# Autodesk Inventor assembly: robot_2016
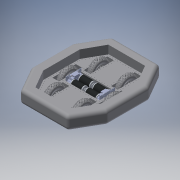
[picture p0: Inventor's stored thumbnail of the model, 180x180]
Saved by Autodesk Inventor 2016 (Build 200138000, 138)
## iProperties
Created: 2016-02-01
Part Number: robot_2016
Document SubType Name: Assembly
Designer: Mentor1102
Sending System: CREO PARAMETRIC BY PTC INC, 2014440
Preprocessor: CREO PARAMETRIC BY PTC INC, 2014440
Title: ROBOT2_ASM
Author: folkj_000
Revision Number: 24LAST_VERSION
## Documents named in this file (52)
- C:\Users\Mentor1102\Desktop\4901 CAD\RobotBase2016\robot_2016.iam
- C:\Users\Mentor1102\Desktop\4901 CAD\RobotBase2016\TOP_PLATE2_AF0.ipt
- C:\Users\Mentor1102\Desktop\4901 CAD\RobotBase2016\MOTORMOUNTBAR_AF0.ipt
- C:\Users\Mentor1102\Desktop\4901 CAD\RobotBase2016\MOTORMOUNTBAR_AF1.ipt
- C:\Users\Mentor1102\Desktop\4901 CAD\RobotBase2016\217-2642-STEP-20140807_AF0.ipt
- C:\Users\Mentor1102\Desktop\4901 CAD\RobotBase2016\217-2642-STEP-20140807_AF1.ipt
- C:\Users\Mentor1102\Desktop\4901 CAD\RobotBase2016\FR8ZZ_HEX_BEARING_1_AF0.ipt
- C:\Users\Mentor1102\Desktop\4901 CAD\RobotBase2016\FR8ZZ_HEX_BEARING_1_AF1.ipt
- C:\Users\Mentor1102\Desktop\4901 CAD\RobotBase2016\PNEUMATIC_WHEEL_AF0_ASM.iam
- C:\Users\Mentor1102\Desktop\4901 CAD\RobotBase2016\AM-1305_500_HEX_SPACER_1_AF0.ipt
- C:\Users\Mentor1102\Desktop\4901 CAD\RobotBase2016\217-2642-STEP-20140807_AF2.ipt
- C:\Users\Mentor1102\Desktop\4901 CAD\RobotBase2016\FR8ZZ_HEX_BEARING_1_AF2.ipt
- C:\Users\Mentor1102\Desktop\4901 CAD\RobotBase2016\FR8ZZ_HEX_BEARING_1_AF3.ipt
- C:\Users\Mentor1102\Desktop\4901 CAD\RobotBase2016\PNEUMATIC_WHEEL_AF1_ASM.iam
- C:\Users\Mentor1102\Desktop\4901 CAD\RobotBase2016\AM-1305_500_HEX_SPACER_1_AF1.ipt
- C:\Users\Mentor1102\Desktop\4901 CAD\RobotBase2016\217-2642-STEP-20140807_AF3.ipt
- C:\Users\Mentor1102\Desktop\4901 CAD\RobotBase2016\PNEUMATIC_WHEEL_AF2_ASM.iam
- C:\Users\Mentor1102\Desktop\4901 CAD\RobotBase2016\AM-1305_500_HEX_SPACER_1_AF2.ipt
- C:\Users\Mentor1102\Desktop\4901 CAD\RobotBase2016\217-2642-STEP-20140807_AF4.ipt
- C:\Users\Mentor1102\Desktop\4901 CAD\RobotBase2016\3X1_9_AF0.ipt
- C:\Users\Mentor1102\Desktop\4901 CAD\RobotBase2016\3X1_9_AF1.ipt
- C:\Users\Mentor1102\Desktop\4901 CAD\RobotBase2016\217-2642-STEP-20140807_AF5.ipt
- C:\Users\Mentor1102\Desktop\4901 CAD\RobotBase2016\217-2642-STEP-20140807_AF6.ipt
- C:\Users\Mentor1102\Desktop\4901 CAD\RobotBase2016\FR8ZZ_HEX_BEARING_1_AF4.ipt
- C:\Users\Mentor1102\Desktop\4901 CAD\RobotBase2016\FR8ZZ_HEX_BEARING_1_AF5.ipt
- C:\Users\Mentor1102\Desktop\4901 CAD\RobotBase2016\PNEUMATIC_WHEEL_AF3_ASM.iam
- C:\Users\Mentor1102\Desktop\4901 CAD\RobotBase2016\AM-1305_500_HEX_SPACER_1_AF3.ipt
- C:\Users\Mentor1102\Desktop\4901 CAD\RobotBase2016\217-2642-STEP-20140807_AF7.ipt
- C:\Users\Mentor1102\Desktop\4901 CAD\RobotBase2016\FR8ZZ_HEX_BEARING_1_AF6.ipt
- C:\Users\Mentor1102\Desktop\4901 CAD\RobotBase2016\FR8ZZ_HEX_BEARING_1_AF7.ipt
- C:\Users\Mentor1102\Desktop\4901 CAD\RobotBase2016\PNEUMATIC_WHEEL_AF4_ASM.iam
- C:\Users\Mentor1102\Desktop\4901 CAD\RobotBase2016\AM-1305_500_HEX_SPACER_1_AF4.ipt
- C:\Users\Mentor1102\Desktop\4901 CAD\RobotBase2016\217-2642-STEP-20140807_AF8.ipt
- C:\Users\Mentor1102\Desktop\4901 CAD\RobotBase2016\PNEUMATIC_WHEEL_AF5_ASM.iam
- C:\Users\Mentor1102\Desktop\4901 CAD\RobotBase2016\AM-1305_500_HEX_SPACER_1_AF5.ipt
- C:\Users\Mentor1102\Desktop\4901 CAD\RobotBase2016\217-2642-STEP-20140807_AF9.ipt
- C:\Users\Mentor1102\Desktop\4901 CAD\RobotBase2016\BAR2_18IN_AF0.ipt
- C:\Users\Mentor1102\Desktop\4901 CAD\RobotBase2016\BAR2_18IN_AF1.ipt
- C:\Users\Mentor1102\Desktop\4901 CAD\RobotBase2016\BAR1_AF0.ipt
- C:\Users\Mentor1102\Desktop\4901 CAD\RobotBase2016\BAR1_AF1.ipt
- C:\Users\Mentor1102\Desktop\4901 CAD\RobotBase2016\BAR6_FRONT_AF0.ipt
- C:\Users\Mentor1102\Desktop\4901 CAD\RobotBase2016\BAR1_AF2.ipt
- C:\Users\Mentor1102\Desktop\4901 CAD\RobotBase2016\BAR1_AF3.ipt
- C:\Users\Mentor1102\Desktop\4901 CAD\RobotBase2016\BAR6_FRONT_AF1.ipt
- C:\Users\Mentor1102\Desktop\4901 CAD\RobotBase2016\BAR_12_AF0.ipt
- C:\Users\Mentor1102\Desktop\4901 CAD\RobotBase2016\BAR_12_AF1.ipt
- C:\Users\Mentor1102\Desktop\4901 CAD\RobotBase2016\3X1_9_AF2.ipt
- C:\Users\Mentor1102\Desktop\4901 CAD\RobotBase2016\3X1_9_AF3.ipt
- C:\Users\Mentor1102\Desktop\4901 CAD\RobotBase2016\BOTTOM_PLATE_AF0.ipt
- C:\Users\Mentor1102\Desktop\5632 CAD\Toughbox Mini.iam
- C:\Users\Mentor1102\Desktop\4901 CAD\Bumpers.ipt
- C:\Users\Mentor1102\Desktop\4901 CAD\Shafts.ipt
## Components (55 placed, 51 different names)
1. 0
2. 1 — Insert:5
3. 2 — Insert:6
4. 36
5. 37
6. 38 — Insert:9
7. 39 — Insert:14
8. 51 [sub-assembly]
9. 52
10. 54
11. 55 — Insert:10
12. 56 — Insert:13
13. 68 [sub-assembly]
14. 69
15. 71
16. 83 [sub-assembly]
17. 84
18. 85
19. 86 — Insert:14
20. 87 — Insert:13
21. 121
22. 122
23. 123 — Insert:7
24. 124 — Insert:11
25. 136 [sub-assembly]
26. 137
27. 139
28. 140 — Insert:8
29. 141 — Insert:12
30. 153 [sub-assembly]
31. 154
32. 156
33. 168 [sub-assembly]
34. 169
35. 170
36. 171 — Mate:1, Flush:1
37. 172
38. 173
39. 174
40. 175 — Mate:2, Mate:3
41. 176
42. 177
43. 178
44. 179
45. 180
46. 181 — Insert:11
47. 182 — Insert:12
48. 183
49. Toughbox Mini:1 [sub-assembly] — Insert:5
50. Toughbox Mini:2 [sub-assembly] — Insert:6
51. Bumpers:1 — Mate:1, Mate:2, Mate:3
52. Shafts:1 — Insert:8
53. Shafts:2 — Insert:9
54. Shafts:3 — Insert:7
55. Shafts:4 — Insert:10
## Relationships (14: Insert 10, Mate 3, Flush 1)
- Insert:5: 1 ↔ Toughbox Mini:1
- Insert:6: 2 ↔ Toughbox Mini:2
- Mate:1: 171 ↔ Bumpers:1
- Mate:2: 175 ↔ Bumpers:1
- Mate:3 (6.35 mm): 175 ↔ Bumpers:1
- Insert:7: 123 ↔ Shafts:3
- Insert:8: 140 ↔ Shafts:1
- Insert:9: 38 ↔ Shafts:2
- Insert:10: 55 ↔ Shafts:4
- Flush:1 (69.85 mm): 171
- Insert:11: 124 ↔ 181
- Insert:12: 141 ↔ 182
- Insert:13: 56 ↔ 87
- Insert:14: 39 ↔ 86
